# Autodesk Inventor assembly: CASE
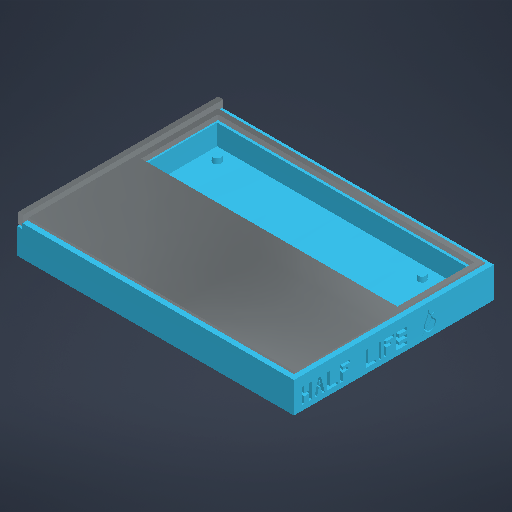
[picture p0: Inventor's stored thumbnail of the model, 512x512]
Saved by Autodesk Inventor 2027.1 (Build 311270010, 270A)
## iProperties
Created: 2026-10-08
Part Number: CASE
Document SubType Name: Assembly
Designer: Richard
Author: Richard
## Documents named in this file (3)
- C:\Users\Richard\Documents\GitHub\HalfLife-Week1\Case\CASE.iam
- C:\Users\Richard\Documents\GitHub\HalfLife-Week1\Case\Lid.ipt
- C:\Users\Richard\Documents\GitHub\HalfLife-Week1\Case\BasePlate.ipt
## Components (2 placed, 2 different names)
1. Lid:1 — Mate:1
2. BasePlate:1 — Mate:1
## Relationships (1: Mate 1)
- Mate:1: Lid:1 ↔ BasePlate:1
## Named parameters: Finish1_Area = 225.398, Finish2_Area = 112.8, Finish2_Thickness = 0.05 mm, Finish3_Area = 112.8, Finish3_Thickness = 0.008 mm, Finish4_Area = 250.061, Finish4_Thickness = 0.012 mm
note: some values were not read from the file. Shown as the stored number, unit unknown: "Finish1_Area", "Finish2_Area", "Finish3_Area", "Finish4_Area".
